# Autodesk Inventor assembly: Mini sumô definitivo Montado
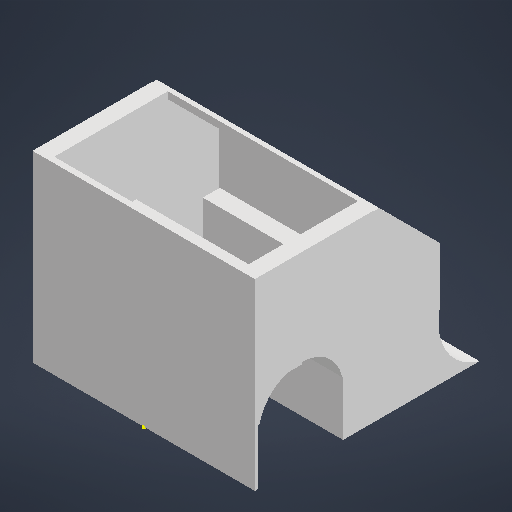
[picture p0: Inventor's stored thumbnail of the model, 512x512]
Saved by Autodesk Inventor 2026.1 (Build 301233000, 233)
## iProperties
Created: 2025-12-07
Part Number: Mini sumô definitivo Montado
Document SubType Name: Assembly
Designer: panto
Author: panto
## Documents named in this file (3)
- C:\Users\panto\OneDrive\Documentos\Inventor\MINI SUMÔ GEAR 2025 - EQUIPE 2\Mini sumô definitivo Montado.iam
- C:\Users\panto\OneDrive\Documentos\Inventor\MINI SUMÔ GEAR 2025 - EQUIPE 2\Mini Sumô Definitivo - TAMPA.ipt
- C:\Users\panto\OneDrive\Documentos\Inventor\MINI SUMÔ GEAR 2025 - EQUIPE 2\Mini Sumô Definitivo - CHASSI.ipt
## Components (2 placed, 2 different names)
1. Mini Sumô Definitivo - TAMPA:1 — Coincidente:1
2. Mini Sumô Definitivo - CHASSI:1 — Coincidente:1
## Relationships (1: Mate 1)
- Coincidente:1 [Mate]: Mini Sumô Definitivo - TAMPA:1 ↔ Mini Sumô Definitivo - CHASSI:1
